# Autodesk Inventor assembly: left_hand_joystick_cam
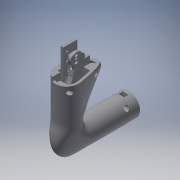
[picture p0: Inventor's stored thumbnail of the model, 180x180]
Saved by Autodesk Inventor 2018 (Build 220112000, 112)
## iProperties
Created: 2018-03-20
Part Number: left_hand_joystick_cam
Document SubType Name: Assembly
Designer: oechslin
Author: oechslin
## Documents named in this file (9)
- C:\Users\oechslin\Documents\Inventor_workspace\20180314_pilot_steeringwheel_design\cam\left_hand_joystick_cam.iam
- C:\Users\oechslin\Documents\Inventor_workspace\20180314_pilot_steeringwheel_design\cam\Palm_pad.ipt
- C:\Users\oechslin\Documents\Inventor_workspace\20180314_pilot_steeringwheel_design\cam\Motor_plate.ipt
- C:\Users\oechslin\Documents\Inventor_workspace\20180314_pilot_steeringwheel_design\cam\Cover.ipt
- C:\Users\oechslin\Documents\Inventor_workspace\20180314_pilot_steeringwheel_design\cam\Base.ipt
- C:\Users\oechslin\Documents\Inventor_workspace\20180314_pilot_steeringwheel_design\cam\Spring_plate.ipt
- C:\Users\oechslin\Documents\Inventor_workspace\20180314_pilot_steeringwheel_design\cam\Rotation_L_2.ipt
- C:\Users\oechslin\Documents\Inventor_workspace\20180314_pilot_steeringwheel_design\cam\Rotation_cam.ipt
- C:\Users\oechslin\Documents\Inventor_workspace\20180314_pilot_steeringwheel_design\cam\joystick_plate.ipt
## Components (9 placed, 8 different names)
1. Palm_pad:1
2. Motor_plate:1
3. Cover:1 — Flush:1, Flush:2, Flush:3
4. Base:1
5. Spring_plate:1
6. Rotation_L_2:1
7. Spring_plate:1
8. Rotation_cam:1
9. joystick_plate:1 — Flush:1, Flush:2, Flush:3
## Relationships (3: Flush 3)
- Flush:1: Cover:1 ↔ joystick_plate:1
- Flush:2: Cover:1 ↔ joystick_plate:1
- Flush:3: Cover:1 ↔ joystick_plate:1
